# Autodesk Inventor assembly: Analogmodul Baugruppe
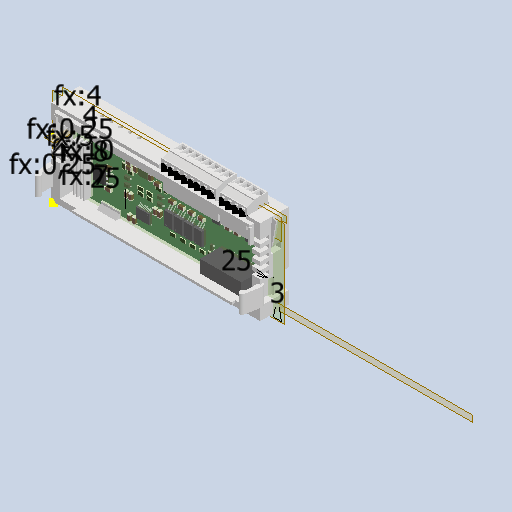
[picture p0: Inventor's stored thumbnail of the model, 512x512]
Saved by Autodesk Inventor 2025.2 (Build 292293000, 293)
## iProperties
Created: 2025-11-01
Part Number: Analogmodul Baugruppe
Document SubType Name: Assembly
Designer: leowa
Author: leowa
## Documents named in this file (6)
- C:\Users\leowa\OneDrive - Fachhochschule Aachen\FH\8. Semester\CAN Tram CAD\Module\Analogmodul Baugruppe.iam
- C:\Users\leowa\OneDrive - Fachhochschule Aachen\FH\8. Semester\CAN Tram CAD\Gehäuse\Generisches Gehäuse V2.ipt
- C:\Users\leowa\OneDrive - Fachhochschule Aachen\FH\8. Semester\CAN Tram CAD\Gehäuse\Analogmodul Gehäuse Deckel.ipt
- C:\Users\leowa\OneDrive - Fachhochschule Aachen\FH\8. Semester\CAN Tram CAD\Platinen\Analogmodul\Analogmodul.iam
- C:\Users\leowa\OneDrive - Fachhochschule Aachen\FH\8. Semester\CAN Tram CAD\Kaufteile\Terminalstecker 4fach\0395000004.iam
- C:\Users\leowa\OneDrive - Fachhochschule Aachen\FH\8. Semester\CAN Tram CAD\Kaufteile\Terminalstecker 8fach\0395000008.iam
## Components (5 placed, 5 different names)
1. Generisches Gehäuse V2:1 — Passend:1, Passend:2, Passend:3, Fluchtend:1, Fluchtend:2, Passend:4
2. Analogmodul Gehäuse Deckel:1 — Fluchtend:1, Fluchtend:2, Passend:4
3. Analogmodul:1 [sub-assembly] — Passend:1, Passend:2, Passend:3, Passend:5, Passend:6, Passend:7, Passend:8
4. 0395000004:1 [sub-assembly] — Passend:5, Passend:8
5. 0395000008:1 [sub-assembly] — Passend:6, Passend:7
## Relationships (10: Mate 8, Flush 2)
- Passend:1 [Mate]: Generisches Gehäuse V2:1 ↔ Analogmodul:1
- Passend:2 [Mate]: Generisches Gehäuse V2:1 ↔ Analogmodul:1
- Passend:3 [Mate] (1 mm): Generisches Gehäuse V2:1 ↔ Analogmodul:1
- Fluchtend:1 [Flush]: Generisches Gehäuse V2:1 ↔ Analogmodul Gehäuse Deckel:1
- Fluchtend:2 [Flush]: Generisches Gehäuse V2:1 ↔ Analogmodul Gehäuse Deckel:1
- Passend:4 [Mate]: Generisches Gehäuse V2:1 ↔ Analogmodul Gehäuse Deckel:1
- Passend:5 [Mate]: Analogmodul:1 ↔ 0395000004:1
- Passend:6 [Mate]: Analogmodul:1 ↔ 0395000008:1
- Passend:7 [Mate]: Analogmodul:1 ↔ 0395000008:1
- Passend:8 [Mate]: Analogmodul:1 ↔ 0395000004:1
